# Autodesk Inventor assembly: tetrix_739083_2012
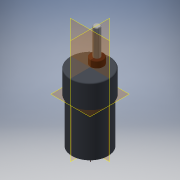
[picture p0: Inventor's stored thumbnail of the model, 180x180]
Saved by Autodesk Inventor 2016 (Build 200138000, 138)
## iProperties
Created: 2015-08-29
Part Number: tetrix_739083_2012
Description: DC Drive Motor
Document SubType Name: Assembly
Designer: PTC
Sending System: Creo  TM  2.0  (c) 2012
PROJECT: FTC
Author: phi
## Documents named in this file (3)
- C:\Users\Tim\Documents\GitHub\phi_robotics\3d-models\FTC_Tetrix_KOP_Block_Party\Tetrix_Kit_FTC\Autodesk Inventor Files\tetrix_motor.iam
- C:\Users\Tim\Documents\GitHub\phi_robotics\3d-models\FTC_Tetrix_KOP_Block_Party\Tetrix_Kit_FTC\Autodesk Inventor Files\tetrix_motor_shell.ipt
- C:\Users\Tim\Documents\GitHub\phi_robotics\3d-models\FTC_Tetrix_KOP_Block_Party\Tetrix_Kit_FTC\Autodesk Inventor Files\tetrix_motor_axle.ipt
## Components (2 placed, 2 different names)
1. TETRIX_739083_MOTOR_2012 — Rotational:1
2. TETRIX_739083_AXLE_2012 — Rotational:1
## Relationships (1: RevoluteJoint 1)
- Rotational:1 [RevoluteJoint]: TETRIX_739083_MOTOR_2012 ↔ TETRIX_739083_AXLE_2012
